# Autodesk Inventor assembly: Adjustable legs
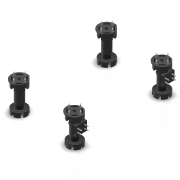
[picture p0: Inventor's stored thumbnail of the model, 180x180]
Saved by Autodesk Inventor 2024 (Build 280153000, 153)
## iProperties
RuleStatus: InUse
AfterAnyParamChange0: PassParameters
AfterAnyUserParamChange0: PassParameters
Created: 2023-03-05
Part Number: Adjustable legs
Document SubType Name: Assembly
Designer: sauliusd
Author: sauliusd
## Documents named in this file (5)
- C:\W4INV 2024 Design\SMART HARDWARE\Legs\Adjustable Legs\Adjustable legs.iam
- C:\W4INV 2024 Design\SMART HARDWARE\Legs\Adjustable Legs\Parts\Legs Skeleton.ipt
- C:\W4INV 2022 Design\LIBRARY\Supports and legs\Legs\ADJUSTABLE LEG.ipt
- C:\W4INV 2024 Design\_LIBRARY\Supports and legs\Legs\ADJUSTABLE LEG\Adjustable leg  BT18 clip included.ipt
- C:\W4INV 2024 Design\_LIBRARY\Supports and legs\Legs\ADJUSTABLE LEG\Adjustable leg  BT18.ipt
## Components (5 placed, 5 different names)
1. @Skeleton — Flush:1, Flush:2, Flush:3, Insert:1, Insert:2
2. Adjustable Leg Front — Insert:1, Angle:1
3. Adjustable leg  BT18 clip included:2
4. Adjustable Leg Back — Insert:2
5. Adjustable leg  BT18:4
## Component patterns: (2 elements, first: Adjustable Leg Front), (2 elements, first: Adjustable Leg Back)
## Relationships (6: Flush 3, Insert 2, Angle 1)
- Flush:1: @Skeleton
- Flush:2: @Skeleton
- Flush:3: @Skeleton
- Insert:1: @Skeleton ↔ Adjustable Leg Front
- Angle:1 (0 deg): Adjustable Leg Front
- Insert:2: @Skeleton ↔ Adjustable Leg Back
## Named parameters: Length = 400 mm, Depth = 300 mm, Shift_X = 0 mm, Shift_Y = -10 mm, Margins_X = 50 mm, Margins_Y = 50 mm, Board_T = 18 mm, Count = 2
